# Autodesk Inventor assembly: SCSNAWJ10-13
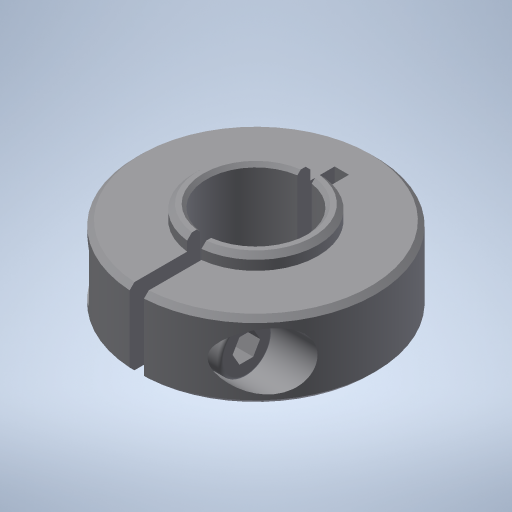
[picture p0: Inventor's stored thumbnail of the model, 512x512]
Saved by Autodesk Inventor 2024.1 (Build 281209000, 209)
## iProperties
Created: 2023-04-15
Part Number: SCSNAWJ10-13
Catalog Web Link: www.cadenas.de
Description: SCBNJ, PSCBNJ, SSCBNJ, SCSNAJ, SCSNAWJ, SCLSJ, PSCLSJ, SSCLSJ-Set Collars - For Bearing Fixing - (For Space Saving) - Slit Compact Type
Vendor: MISUMI
Document SubType Name: Assembly
Designer: psAdmin
Manufacturer: MISUMI
Mass: 3.10884 g
Surface Area: 22.2867 cm^2
Volume: 3.10884 cm^3
Density: 1 g/cm^3
Category: PARTsolutions
Company: MISUMI
PSOL_IDENT_0: {$CADENAS_DATA/23d-libs/misumi/metric/03_set_collars/scbnj_asmtab.prj},249 {VTYP=3D},{STYP=ASSTAB},{
PSOL_IDENT_1: NB=SCSNAWJ10-13},{LINA=SCSNAWJ10-13},{NN=SCBNJ, PSCBNJ, SSCBNJ, SCSNAJ, SCSNAWJ, SCLSJ, PSCLSJ, SSCL
PSOL_IDENT_2: SJ},{DATE=30.06.2021 12:51:49},{GEOMDATE=14.06.2021 09:12:30},{VERSION=},{LINEID=60},{WBVAR=TS,MAT,S
PSOL_IDENT_3: T,DSS},{WBNUMERIC=DSS}  {NB=SCSNAWJ10-13},{LINA=SCSNAWJ10-13},{KT=DUMMY},{PN=SCSNAWJ10-13},{TYPE=SCS
PSOL_IDENT_4: NAWJ},{D=10},{TS=SN},{TS1='SN','Short Nose','LN','Long Nose'},{MAT=2017},{MATA='1045','1045 Carbon S
PSOL_IDENT_5: teel','304','304 Stainless Steel','2017','2017 Aluminum Alloy'},{ST=Clear Anodize},{ST0='-','-','Cle
PSOL_IDENT_6: ar Anodize','Clear Anodize'},{DSS=13},{DS1=13,14},{AC=Hexagon Socket Head Cap Screw 1 Pc. (SUS)},{AB=
PSOL_IDENT_7: 6800ZZ(19)},{B=9.5},{B11=9.5},{B1=0},{B12=12},{D1=25},{M=M3},{THMD=3},{BB=8},{C=0.5},{L=10},{DD=3.5}
PSOL_IDENT_8: ,{R=3.00},{W=1.5},{X=8.0},{Y=4},{Z=9.0},{PPATH=scbnj_templ.prj},{TIFF=1}
NB: SCSNAWJ10-13
NN: SCBNJ, PSCBNJ, SSCBNJ, SCSNAJ, SCSNAWJ, SCLSJ, PSCLSJ, SSCLSJ
NT: Set Collars - For Bearing Fixing - (For Space Saving) - Slit Compact Type
NBSYN: $PN.
LINA: SCSNAWJ10-13
CATALOG: Misumi
PN: SCSNAWJ10-13
D: 10
TS: Short Nose
MAT: 2017 Aluminum Alloy
ST: Clear Anodize
DSS: 13
AC: Hexagon Socket Head Cap Screw 1 Pc. (SUS)
AB: 6800ZZ(19)
B: 9.5
B1: 0
D1: 25
M: M3
BB: 8
DD: 3.5
R: 3
W: 1.5
X: 8
Y: 4
Z: 9
SUPPLIER: MISUMI
ARTICLENO: SCSNAWJ10-13
BOMINFO: SCSNAWJ10-13
CREATOR: CADENAS GmbH
Title: SCSNAWJ10-13
Author: Cadenas PARTsolutions
Comments: Set Collars - For Bearing Fixing - (For Space Saving) - Slit Compact Type
## Documents named in this file (3)
- C:\Users\haruy\OneDrive - Kyushu University\cad\000_parts\セットカラー\AIS2022\SCSNAWJ10-13.iam
- C:\Users\haruy\OneDrive - Kyushu University\cad\000_parts\セットカラー\AIS2022\SCSNAWJ10-13b.ipt
- C:\Users\haruy\OneDrive - Kyushu University\cad\000_parts\セットカラー\AIS2022\Slotted head cap screw ISO 4762 - M3x10.ipt
## Components (2 placed, 2 different names)
1. SCSNAWJ10-13b:1 — body_screw_Z@1 <-> IP4_Z@2
2. Slotted head cap screw ISO 4762 - M3x10:1 — body_screw_Z@1 <-> IP4_Z@2
## Relationships (1: Mate 1)
- body_screw_Z@1 <-> IP4_Z@2 [Mate]: SCSNAWJ10-13b:1 ↔ Slotted head cap screw ISO 4762 - M3x10:1
